# Autodesk Inventor assembly: ASY NDM-VOS_powder_hopper
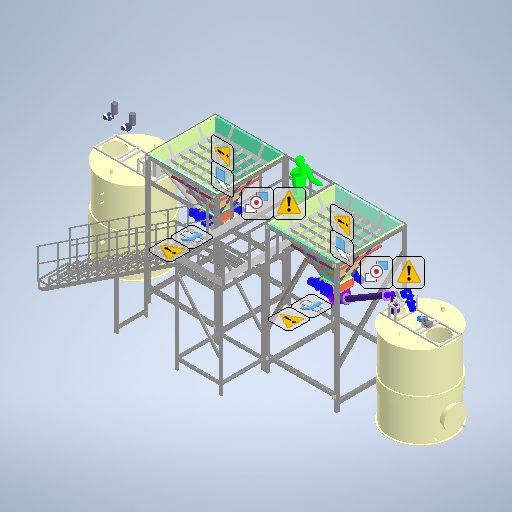
[picture p0: Inventor's stored thumbnail of the model, 512x512]
Saved by Autodesk Inventor 2025 (Build 290162010, 162A)
## iProperties
Created: 2024-07-24
Part Number: ASY NDM-VOS_powder_hopper
Document SubType Name: Assembly
Designer: admin
Author: admin
## Documents named in this file (31)
- C:\Users\pokla\Documents\Inventor\NDM-VOS_powder_hopper\ASY NDM-VOS_powder_hopper.iam
- C:\Users\pokla\Documents\Inventor\NDM-VOS_powder_hopper\human 01\ч ASY human dummy 01.iam
- C:\Users\pokla\Documents\Inventor\NDM-VOS_powder_hopper\NDM-VOS dummy3.ipt
- C:\Users\pokla\Documents\Inventor\NDM-VOS_powder_hopper\NDM-VOS dummy FLOOR.ipt
- C:\Users\pokla\Documents\Inventor\NDM-VOS_powder_hopper\NDM-VOS dummy Crane.ipt
- C:\Users\pokla\Documents\Inventor\NDM-VOS_powder_hopper\NDM-VOS dummy upstairse.ipt
- C:\Users\pokla\Documents\Inventor\NDM-VOS_powder_hopper\Workspaces\Workspace\Cone\ASY MSC 100 cone.iam
- C:\Users\pokla\Documents\Inventor\NDM-VOS_powder_hopper\ASY HPR 200  Frame.iam
- C:\Users\pokla\Documents\Inventor\NDM-VOS_powder_hopper\TM06198C pump.ipt
- C:\Users\pokla\Documents\Inventor\NDM-VOS_powder_hopper\ASY стойка.iam
- C:\Users\pokla\Documents\Inventor\NDM-VOS_powder_hopper\ASY NVPH-400 shredder.iam
- C:\Users\user\YandexDisk-badmisterfox\домашниий пк\Inventor\Content Center Files\en-US\ISO 4775\ISO 4775 - M12.ipt
- C:\Users\pokla\Documents\Inventor\NDM-VOS_powder_hopper\ASY NVPH-300 hopper.iam
- C:\Users\pokla\Documents\Inventor\NDM-VOS_powder_hopper\ASY Augur motor frame 500.iam
- C:\Users\pokla\Documents\Inventor\NDM-VOS_powder_hopper\3d party\motor-reductor NMRV040\motor-reductor NMRV040.iam
- C:\Users\pokla\Documents\Inventor\NDM-VOS_powder_hopper\3d party\Mixer 22.04.24\ASY mixer 3.iam
- C:\Users\pokla\Documents\Inventor\NDM-VOS_powder_hopper\NDM-VOS 777 sredder wall 7.ipt
- C:\Users\pokla\Documents\Inventor\NDM-VOS_powder_hopper\NDM-VOS 778 engine plate.ipt
- C:\Users\pokla\Documents\Inventor\NDM-VOS_powder_hopper\3d party\PCRV071-063SHFA_MS71B5\PCRV071-063SHFA_MS71B5\PCRV071-063SHFA_MS71B5.ipt
- C:\Users\pokla\Documents\Inventor\NDM-VOS_powder_hopper\NDM-VOS 712 flange.ipt
- C:\Users\pokla\Documents\Inventor\NDM-VOS_powder_hopper\NDM-VOS 913 flange bolt.ipt
- C:\Users\pokla\Documents\Inventor\NDM-VOS_powder_hopper\NDM-VOS 715 flange.ipt
- C:\Users\pokla\Documents\Inventor\NDM-VOS_powder_hopper\FL3.6.2  Motor pillar.ipt
- C:\Users\pokla\Documents\Inventor\NDM-VOS_powder_hopper\ASY платформа.iam
- C:\Users\pokla\Documents\Inventor\NDM-VOS_powder_hopper\ASY Рама №1 платформа.iam
- C:\Users\pokla\Documents\Inventor\NDM-VOS_powder_hopper\ASY Рама №2 платформа.iam
- C:\Users\pokla\Documents\Inventor\NDM-VOS_powder_hopper\ASY Рама №3 платформа.iam
- C:\Users\pokla\Documents\Inventor\NDM-VOS_powder_hopper\ASY Лестница.iam
- C:\Users\pokla\Documents\Inventor\NDM-VOS_powder_hopper\ASY Лестница перила.iam
- C:\Users\pokla\Documents\Inventor\NDM-VOS_powder_hopper\ISO 4019 - 80x40x2 - 1090.ipt
- C:\Users\pokla\Documents\Inventor\NDM-VOS_powder_hopper\NDM-VOS Пятка под стойки.ipt
## Components (52 placed, 30 different names)
1. NDM-VOS dummy3:2 — Mate:6, Mate:8, Mate:9, Mate:60
2. ч ASY human dummy 01:1 [sub-assembly]
3. NDM-VOS dummy FLOOR:1 — Mate:5, Mate:6, Mate:8, Mate:10, Mate:18
4. NDM-VOS dummy Crane:1 — Mate:10
5. NDM-VOS dummy upstairse:1 — Mate:18
6. ASY MSC 100 CONE:1 [sub-assembly] — Mate:20, Rigid:27, Mate:35, Mate:36
7. ASY HPR 200  Frame:1 [sub-assembly] — Mate:20, Mate:35, Mate:36, Flush:45, Flush:46, Mate:56
8. TM06198C pump:1
9. ASY HPR 200  Frame:2 [sub-assembly] — Mate:52, Mate:53, Mate:54, Flush:47, Flush:48, Mate:57
10. ASY стойка:1 [sub-assembly] — Flush:43, Flush:44, Mate:55, Rigid:43, Rigid:44, Flush:45, Flush:46, Mate:56, Flush:47, Flush:48, Mate:57, Rigid:58, Rotational:16
11. ASY стойка:2 [sub-assembly] — Rigid:43, Rigid:56, Rigid:57
12. ASY стойка:3 [sub-assembly] — Rigid:44, Rigid:49, Rigid:50, Rigid:52, Rigid:53
13. ASY MSC 100 CONE:2 [sub-assembly] — Mate:52, Mate:53, Mate:54, Rigid:42
14. TM06198C pump:2
15. ASY NVPH-400 shredder:1 [sub-assembly] — Rigid:27, Mate:31, Mate:32
16. ISO 4775 M12:1 — Mate:31, Mate:32
17. ASY NVPH-300 hopper:1 [sub-assembly] — Rigid:34
18. ASY NVPH-400 shredder:2 [sub-assembly] — Rigid:30, Rigid:42
19. ASY NVPH-300 hopper:2 [sub-assembly] — Rigid:30
20. NDM-VOS dummy3:1 — Mate:5, Mate:9
21. ASY Augur motor frame 500:1 [sub-assembly] — Mate:40, Mate:42, Flush:34, Mate:43, Flush:35, Mate:44, Mate:45, Flush:36, Flush:53
22. motor-reductor NMRV040:1 [sub-assembly] — Rotational:15
23. ASY mixer 3:1 [sub-assembly] — Rotational:15
24. NDM-VOS 112 sredder wall sub:1 — Rigid:34, Rigid:35
25. NDM-VOS 778 engine plate:1 — Rigid:35, Rigid:36, Mate:39, Mate:41
26. PCRV071-063SHFA_MS71B5:1 — Rigid:36
27. NDM-VOS 712 flange:1 — Mate:39, Mate:40, Flush:32, Flush:33
28. NDM-VOS 913 flange bolt:1 — Rigid:37
29. NDM-VOS 913 flange bolt:2 — Rigid:37
30. NDM-VOS 712 flange:2 — Mate:41, Flush:32, Flush:33
31. NDM-VOS 715 flange:1 — Mate:42, Flush:34
32. FL3.6.2  Motor pillar:1 — Mate:43, Flush:35, Mate:44
33. NDM-VOS 715 flange:2 — Mate:45, Flush:36
34. ASY платформа:1 [sub-assembly] — Flush:43, Flush:44, Mate:55, Rigid:45, Rigid:46, Flush:49, Mate:58, Flush:50
35. ASY Рама №1 платформа:1 [sub-assembly] — Rigid:45, Rigid:47, Rigid:48
36. ASY Рама №1 платформа:2 [sub-assembly] — Rigid:46
37. ASY Рама №2 платформа:1 [sub-assembly] — Rigid:47
38. ASY Рама №3 платформа:1 [sub-assembly] — Rigid:48
39. ASY Лестница:1 [sub-assembly] — Flush:49, Mate:58, Flush:50, Mate:59, Flush:51, Flush:52, Rigid:54, Rigid:55
40. ASY Лестница перила:1 [sub-assembly] — Mate:59, Flush:51, Flush:52, Rigid:51
41. ISO 4019 - 80x40x2 - 1090:1 — Rigid:49
42. ISO 4019 - 80x40x2 - 1090:2 — Rigid:50
43. ASY Лестница перила:2 [sub-assembly] — Rigid:51
44. NDM-VOS Пятка под стойки:1 — Rigid:52
45. NDM-VOS Пятка под стойки:2 — Rigid:53
46. NDM-VOS Пятка под стойки:3 — Rigid:54
47. NDM-VOS Пятка под стойки:4 — Rigid:55
48. NDM-VOS Пятка под стойки:5 — Rigid:57
49. NDM-VOS Пятка под стойки:6 — Rigid:56
50. NDM-VOS Пятка под стойки:7 — Rigid:58
51. NDM-VOS Пятка под стойки:8 — Rotational:16
52. ASY Augur motor frame 500:2 [sub-assembly] — Flush:53, Mate:60
## Relationships (76: Mate 30, WeldJoint 24, Flush 20, RevoluteJoint 2)
- Mate:5: NDM-VOS dummy FLOOR:1 ↔ NDM-VOS dummy3:1
- Mate:6: NDM-VOS dummy3:2 ↔ NDM-VOS dummy FLOOR:1
- Mate:8 (1200 mm): NDM-VOS dummy3:2 ↔ NDM-VOS dummy FLOOR:1
- Mate:9 (-1830 mm): NDM-VOS dummy3:2 ↔ NDM-VOS dummy3:1
- Mate:10 (3500 mm): NDM-VOS dummy FLOOR:1 ↔ NDM-VOS dummy Crane:1
- Mate:18: NDM-VOS dummy FLOOR:1 ↔ NDM-VOS dummy upstairse:1
- [Flush]: ASY HPR 200  Frame:1
- Mate:20: ASY MSC 100 CONE:1 ↔ ASY HPR 200  Frame:1
- Rigid:27 [WeldJoint]: ASY MSC 100 CONE:1 ↔ ASY NVPH-400 shredder:1
- [WeldJoint]: ASY NVPH-400 shredder:1 ↔ ASY NVPH-300 hopper:1
- [Mate]: ASY NVPH-400 shredder:1 ↔ ASY NVPH-300 hopper:1
- [Flush]: ASY NVPH-400 shredder:1 ↔ ASY NVPH-300 hopper:1
- Mate:31: ASY NVPH-400 shredder:1 ↔ ISO 4775 M12:1
- Mate:32: ASY NVPH-400 shredder:1 ↔ ISO 4775 M12:1
- [Mate]: ASY NVPH-400 shredder:1 ↔ ASY NVPH-300 hopper:1
- Rigid:30 [WeldJoint]: ASY NVPH-400 shredder:2 ↔ ASY NVPH-300 hopper:2
- [Flush]: NDM-VOS dummy3:1 ↔ ASY Augur motor frame 500:1
- [Mate]: NDM-VOS dummy3:1 ↔ ASY Augur motor frame 500:1
- [Flush]: NDM-VOS dummy3:1 ↔ ASY Augur motor frame 500:1
- Mate:35: ASY MSC 100 CONE:1 ↔ ASY HPR 200  Frame:1
- Mate:36: ASY MSC 100 CONE:1 ↔ ASY HPR 200  Frame:1
- Rotational:15 [RevoluteJoint]: motor-reductor NMRV040:1 ↔ ASY mixer 3:1
- Rigid:34 [WeldJoint]: ASY NVPH-300 hopper:1 ↔ NDM-VOS 112 sredder wall sub:1
- Rigid:35 [WeldJoint]: NDM-VOS 112 sredder wall sub:1 ↔ NDM-VOS 778 engine plate:1
- Rigid:36 [WeldJoint]: NDM-VOS 778 engine plate:1 ↔ PCRV071-063SHFA_MS71B5:1
- Mate:39: NDM-VOS 778 engine plate:1 ↔ NDM-VOS 712 flange:1
- Mate:40 (380 mm): ASY Augur motor frame 500:1 ↔ NDM-VOS 712 flange:1
- Mate:41: NDM-VOS 778 engine plate:1 ↔ NDM-VOS 712 flange:2
- Flush:32: NDM-VOS 712 flange:1 ↔ NDM-VOS 712 flange:2
- Flush:33: NDM-VOS 712 flange:1 ↔ NDM-VOS 712 flange:2
- Mate:42: ASY Augur motor frame 500:1 ↔ NDM-VOS 715 flange:1
- Flush:34: ASY Augur motor frame 500:1 ↔ NDM-VOS 715 flange:1
- Mate:43: ASY Augur motor frame 500:1 ↔ FL3.6.2  Motor pillar:1
- Flush:35: ASY Augur motor frame 500:1 ↔ FL3.6.2  Motor pillar:1
- Mate:44: ASY Augur motor frame 500:1 ↔ FL3.6.2  Motor pillar:1
- Mate:45: ASY Augur motor frame 500:1 ↔ NDM-VOS 715 flange:2
- Flush:36: ASY Augur motor frame 500:1 ↔ NDM-VOS 715 flange:2
- Rigid:37 [WeldJoint]: NDM-VOS 913 flange bolt:1 ↔ NDM-VOS 913 flange bolt:2
- Mate:52: ASY HPR 200  Frame:2 ↔ ASY MSC 100 CONE:2
- Mate:53: ASY HPR 200  Frame:2 ↔ ASY MSC 100 CONE:2
- Mate:54: ASY HPR 200  Frame:2 ↔ ASY MSC 100 CONE:2
- Rigid:42 [WeldJoint]: ASY MSC 100 CONE:2 ↔ ASY NVPH-400 shredder:2
- Flush:43: ASY стойка:1 ↔ ASY платформа:1
- Flush:44: ASY стойка:1 ↔ ASY платформа:1
- Mate:55: ASY стойка:1 ↔ ASY платформа:1
- Rigid:43 [WeldJoint] (1790 mm): ASY стойка:1 ↔ ASY стойка:2
- Rigid:44 [WeldJoint] (2920 mm): ASY стойка:1 ↔ ASY стойка:3
- Rigid:45 [WeldJoint]: ASY платформа:1 ↔ ASY Рама №1 платформа:1
- Rigid:46 [WeldJoint]: ASY платформа:1 ↔ ASY Рама №1 платформа:2
- Rigid:47 [WeldJoint]: ASY Рама №1 платформа:1 ↔ ASY Рама №2 платформа:1
- Rigid:48 [WeldJoint]: ASY Рама №1 платформа:1 ↔ ASY Рама №3 платформа:1
- Flush:45: ASY HPR 200  Frame:1 ↔ ASY стойка:1
- Flush:46: ASY HPR 200  Frame:1 ↔ ASY стойка:1
- Mate:56: ASY HPR 200  Frame:1 ↔ ASY стойка:1
- Flush:47: ASY HPR 200  Frame:2 ↔ ASY стойка:1
- Flush:48: ASY HPR 200  Frame:2 ↔ ASY стойка:1
- Mate:57: ASY HPR 200  Frame:2 ↔ ASY стойка:1
- Flush:49: ASY платформа:1 ↔ ASY Лестница:1
- Mate:58: ASY платформа:1 ↔ ASY Лестница:1
- Flush:50 (40 mm): ASY платформа:1 ↔ ASY Лестница:1
- Rigid:49 [WeldJoint] (-240 mm): ASY стойка:3 ↔ ISO 4019 - 80x40x2 - 1090:1
- Rigid:50 [WeldJoint] (-240 mm): ASY стойка:3 ↔ ISO 4019 - 80x40x2 - 1090:2
- Mate:59: ASY Лестница:1 ↔ ASY Лестница перила:1
- Flush:51 (8.5 mm): ASY Лестница:1 ↔ ASY Лестница перила:1
- Flush:52 (10 mm): ASY Лестница:1 ↔ ASY Лестница перила:1
- Rigid:51 [WeldJoint] (800 mm): ASY Лестница перила:1 ↔ ASY Лестница перила:2
- Rigid:52 [WeldJoint]: ASY стойка:3 ↔ NDM-VOS Пятка под стойки:1
- Rigid:53 [WeldJoint]: ASY стойка:3 ↔ NDM-VOS Пятка под стойки:2
- Rigid:54 [WeldJoint]: ASY Лестница:1 ↔ NDM-VOS Пятка под стойки:3
- Rigid:55 [WeldJoint]: ASY Лестница:1 ↔ NDM-VOS Пятка под стойки:4
- Rigid:56 [WeldJoint]: ASY стойка:2 ↔ NDM-VOS Пятка под стойки:6
- Rigid:57 [WeldJoint]: ASY стойка:2 ↔ NDM-VOS Пятка под стойки:5
- Rigid:58 [WeldJoint]: ASY стойка:1 ↔ NDM-VOS Пятка под стойки:7
- Rotational:16 [RevoluteJoint]: ASY стойка:1 ↔ NDM-VOS Пятка под стойки:8
- Flush:53: ASY Augur motor frame 500:1 ↔ ASY Augur motor frame 500:2
- Mate:60: NDM-VOS dummy3:2 ↔ ASY Augur motor frame 500:2
